# Autodesk Inventor assembly: Corpo2-3
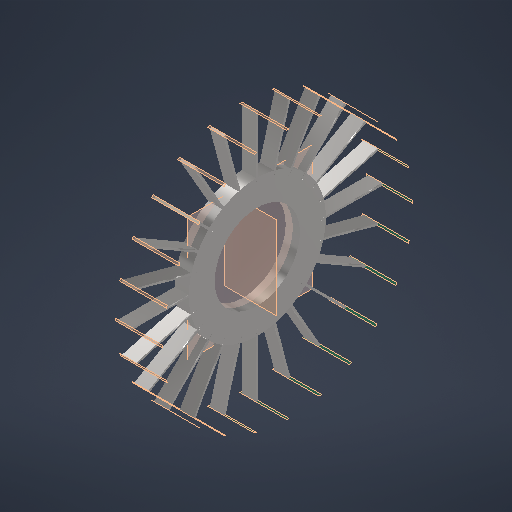
[picture p0: Inventor's stored thumbnail of the model, 512x512]
Saved by Autodesk Inventor 2026.2 (Build 302298010, 298A)
## iProperties
Created: 2026-05-01
Part Number: Corpo2-3
Document SubType Name: Assembly
Designer: Yan
Author: Yan
## Documents named in this file (3)
- C:\Users\Yan\Desktop\Turbina\Corpo2-3.iam
- C:\Users\Yan\Desktop\Turbina\CorpoDiscoPaleSatdio2-3-DimensioniAprossimate.ipt
- C:\Users\Yan\Desktop\Turbina\PalaCorpoStadio2-3.ipt
## Components (25 placed, 2 different names)
1. CorpoDiscoPaleSatdio2-3-DimensioniAprossimate:1 — Mate:1, Mate:2, Mate:3, Mate:4, Mate:5, Mate:6, Mate:7, Mate:8, Mate:9, Mate:10, Mate:11, Mate:12, Mate:13, Mate:14, Mate:15, Mate:16, Mate:17, Mate:18, Mate:19, Mate:20, Mate:21, Mate:22, Mate:23, Mate:24, Mate:25, Mate:26, Mate:27, Mate:28, Mate:29, Mate:30, Mate:31, Mate:32, Mate:33, Mate:34, Mate:35, Mate:36, Mate:37, Mate:38, Mate:39, Mate:40, Mate:41, Mate:42, Mate:43, Mate:44, Mate:45, Mate:46, Mate:47, Mate:48, Mate:49, Mate:50, Mate:51, Flush:1, Flush:2, Flush:3, Flush:4, Flush:5, Flush:6, Flush:7, Flush:8, Flush:9, Flush:10, Flush:11, Flush:12, Flush:13, Flush:14, Flush:15, Flush:16, Flush:17, Flush:18, Flush:19, Flush:20, Flush:21, Flush:22, Flush:23, Flush:24, Flush:25
2. PalaCorpoStadio2-3:1 — Mate:13, Mate:48, Flush:21
3. PalaCorpoStadio2-3:2 — Mate:14, Mate:47, Flush:22
4. PalaCorpoStadio2-3:3 — Mate:15, Mate:46, Flush:23
5. PalaCorpoStadio2-3:4 — Mate:16, Mate:45, Flush:24
6. PalaCorpoStadio2-3:5 — Mate:17, Mate:44, Flush:17
7. PalaCorpoStadio2-3:6 — Mate:18, Mate:43, Flush:16
8. PalaCorpoStadio2-3:7 — Mate:19, Mate:39, Flush:14
9. PalaCorpoStadio2-3:8 — Mate:20, Mate:40, Flush:15
10. PalaCorpoStadio2-3:9 — Mate:21, Mate:38, Flush:12
11. PalaCorpoStadio2-3:10 — Mate:22, Mate:37, Flush:11
12. PalaCorpoStadio2-3:11 — Mate:41, Mate:42, Flush:13
13. PalaCorpoStadio2-3:12 — Mate:23, Mate:36, Flush:10
14. PalaCorpoStadio2-3:13 — Mate:1, Mate:34, Flush:8
15. PalaCorpoStadio2-3:14 — Mate:2, Mate:32, Flush:6
16. PalaCorpoStadio2-3:15 — Mate:3, Mate:33, Flush:7
17. PalaCorpoStadio2-3:16 — Mate:4, Mate:35, Flush:9
18. PalaCorpoStadio2-3:17 — Mate:5, Mate:31, Flush:5
19. PalaCorpoStadio2-3:18 — Mate:6, Mate:30, Flush:4
20. PalaCorpoStadio2-3:19 — Mate:7, Mate:29, Flush:3
21. PalaCorpoStadio2-3:20 — Mate:8, Mate:24, Flush:2
22. PalaCorpoStadio2-3:21 — Mate:9, Mate:25, Flush:1, Flush:25
23. PalaCorpoStadio2-3:22 — Mate:10, Mate:26, Mate:51, Flush:18
24. PalaCorpoStadio2-3:23 — Mate:11, Mate:27, Mate:50, Flush:19
25. PalaCorpoStadio2-3:24 — Mate:12, Mate:28, Mate:49, Flush:20
## Relationships (76: Mate 51, Flush 25)
- Mate:1: CorpoDiscoPaleSatdio2-3-DimensioniAprossimate:1 ↔ PalaCorpoStadio2-3:13
- Mate:2: CorpoDiscoPaleSatdio2-3-DimensioniAprossimate:1 ↔ PalaCorpoStadio2-3:14
- Mate:3: CorpoDiscoPaleSatdio2-3-DimensioniAprossimate:1 ↔ PalaCorpoStadio2-3:15
- Mate:4: CorpoDiscoPaleSatdio2-3-DimensioniAprossimate:1 ↔ PalaCorpoStadio2-3:16
- Mate:5: CorpoDiscoPaleSatdio2-3-DimensioniAprossimate:1 ↔ PalaCorpoStadio2-3:17
- Mate:6: CorpoDiscoPaleSatdio2-3-DimensioniAprossimate:1 ↔ PalaCorpoStadio2-3:18
- Mate:7: CorpoDiscoPaleSatdio2-3-DimensioniAprossimate:1 ↔ PalaCorpoStadio2-3:19
- Mate:8: CorpoDiscoPaleSatdio2-3-DimensioniAprossimate:1 ↔ PalaCorpoStadio2-3:20
- Mate:9: CorpoDiscoPaleSatdio2-3-DimensioniAprossimate:1 ↔ PalaCorpoStadio2-3:21
- Mate:10: CorpoDiscoPaleSatdio2-3-DimensioniAprossimate:1 ↔ PalaCorpoStadio2-3:22
- Mate:11: CorpoDiscoPaleSatdio2-3-DimensioniAprossimate:1 ↔ PalaCorpoStadio2-3:23
- Mate:12: CorpoDiscoPaleSatdio2-3-DimensioniAprossimate:1 ↔ PalaCorpoStadio2-3:24
- Mate:13: CorpoDiscoPaleSatdio2-3-DimensioniAprossimate:1 ↔ PalaCorpoStadio2-3:1
- Mate:14: CorpoDiscoPaleSatdio2-3-DimensioniAprossimate:1 ↔ PalaCorpoStadio2-3:2
- Mate:15: CorpoDiscoPaleSatdio2-3-DimensioniAprossimate:1 ↔ PalaCorpoStadio2-3:3
- Mate:16: CorpoDiscoPaleSatdio2-3-DimensioniAprossimate:1 ↔ PalaCorpoStadio2-3:4
- Mate:17: CorpoDiscoPaleSatdio2-3-DimensioniAprossimate:1 ↔ PalaCorpoStadio2-3:5
- Mate:18: CorpoDiscoPaleSatdio2-3-DimensioniAprossimate:1 ↔ PalaCorpoStadio2-3:6
- Mate:19: CorpoDiscoPaleSatdio2-3-DimensioniAprossimate:1 ↔ PalaCorpoStadio2-3:7
- Mate:20: CorpoDiscoPaleSatdio2-3-DimensioniAprossimate:1 ↔ PalaCorpoStadio2-3:8
- Mate:21: CorpoDiscoPaleSatdio2-3-DimensioniAprossimate:1 ↔ PalaCorpoStadio2-3:9
- Mate:22: CorpoDiscoPaleSatdio2-3-DimensioniAprossimate:1 ↔ PalaCorpoStadio2-3:10
- Mate:23: CorpoDiscoPaleSatdio2-3-DimensioniAprossimate:1 ↔ PalaCorpoStadio2-3:12
- Mate:24: CorpoDiscoPaleSatdio2-3-DimensioniAprossimate:1 ↔ PalaCorpoStadio2-3:20
- Mate:25: CorpoDiscoPaleSatdio2-3-DimensioniAprossimate:1 ↔ PalaCorpoStadio2-3:21
- Mate:26: CorpoDiscoPaleSatdio2-3-DimensioniAprossimate:1 ↔ PalaCorpoStadio2-3:22
- Mate:27: CorpoDiscoPaleSatdio2-3-DimensioniAprossimate:1 ↔ PalaCorpoStadio2-3:23
- Mate:28: CorpoDiscoPaleSatdio2-3-DimensioniAprossimate:1 ↔ PalaCorpoStadio2-3:24
- Mate:29: CorpoDiscoPaleSatdio2-3-DimensioniAprossimate:1 ↔ PalaCorpoStadio2-3:19
- Mate:30: CorpoDiscoPaleSatdio2-3-DimensioniAprossimate:1 ↔ PalaCorpoStadio2-3:18
- Mate:31: CorpoDiscoPaleSatdio2-3-DimensioniAprossimate:1 ↔ PalaCorpoStadio2-3:17
- Mate:32: CorpoDiscoPaleSatdio2-3-DimensioniAprossimate:1 ↔ PalaCorpoStadio2-3:14
- Mate:33: CorpoDiscoPaleSatdio2-3-DimensioniAprossimate:1 ↔ PalaCorpoStadio2-3:15
- Mate:34: CorpoDiscoPaleSatdio2-3-DimensioniAprossimate:1 ↔ PalaCorpoStadio2-3:13
- Mate:35: CorpoDiscoPaleSatdio2-3-DimensioniAprossimate:1 ↔ PalaCorpoStadio2-3:16
- Mate:36: CorpoDiscoPaleSatdio2-3-DimensioniAprossimate:1 ↔ PalaCorpoStadio2-3:12
- Mate:37: CorpoDiscoPaleSatdio2-3-DimensioniAprossimate:1 ↔ PalaCorpoStadio2-3:10
- Mate:38: CorpoDiscoPaleSatdio2-3-DimensioniAprossimate:1 ↔ PalaCorpoStadio2-3:9
- Mate:39: CorpoDiscoPaleSatdio2-3-DimensioniAprossimate:1 ↔ PalaCorpoStadio2-3:7
- Mate:40: CorpoDiscoPaleSatdio2-3-DimensioniAprossimate:1 ↔ PalaCorpoStadio2-3:8
- Mate:41: CorpoDiscoPaleSatdio2-3-DimensioniAprossimate:1 ↔ PalaCorpoStadio2-3:11
- Mate:42: CorpoDiscoPaleSatdio2-3-DimensioniAprossimate:1 ↔ PalaCorpoStadio2-3:11
- Mate:43: CorpoDiscoPaleSatdio2-3-DimensioniAprossimate:1 ↔ PalaCorpoStadio2-3:6
- Mate:44: CorpoDiscoPaleSatdio2-3-DimensioniAprossimate:1 ↔ PalaCorpoStadio2-3:5
- Mate:45: CorpoDiscoPaleSatdio2-3-DimensioniAprossimate:1 ↔ PalaCorpoStadio2-3:4
- Mate:46: CorpoDiscoPaleSatdio2-3-DimensioniAprossimate:1 ↔ PalaCorpoStadio2-3:3
- Mate:47: CorpoDiscoPaleSatdio2-3-DimensioniAprossimate:1 ↔ PalaCorpoStadio2-3:2
- Mate:48: CorpoDiscoPaleSatdio2-3-DimensioniAprossimate:1 ↔ PalaCorpoStadio2-3:1
- Mate:49: CorpoDiscoPaleSatdio2-3-DimensioniAprossimate:1 ↔ PalaCorpoStadio2-3:24
- Mate:50: CorpoDiscoPaleSatdio2-3-DimensioniAprossimate:1 ↔ PalaCorpoStadio2-3:23
- Mate:51: CorpoDiscoPaleSatdio2-3-DimensioniAprossimate:1 ↔ PalaCorpoStadio2-3:22
- Flush:1: CorpoDiscoPaleSatdio2-3-DimensioniAprossimate:1 ↔ PalaCorpoStadio2-3:21
- Flush:2: CorpoDiscoPaleSatdio2-3-DimensioniAprossimate:1 ↔ PalaCorpoStadio2-3:20
- Flush:3: CorpoDiscoPaleSatdio2-3-DimensioniAprossimate:1 ↔ PalaCorpoStadio2-3:19
- Flush:4: CorpoDiscoPaleSatdio2-3-DimensioniAprossimate:1 ↔ PalaCorpoStadio2-3:18
- Flush:5: CorpoDiscoPaleSatdio2-3-DimensioniAprossimate:1 ↔ PalaCorpoStadio2-3:17
- Flush:6: CorpoDiscoPaleSatdio2-3-DimensioniAprossimate:1 ↔ PalaCorpoStadio2-3:14
- Flush:7: CorpoDiscoPaleSatdio2-3-DimensioniAprossimate:1 ↔ PalaCorpoStadio2-3:15
- Flush:8: CorpoDiscoPaleSatdio2-3-DimensioniAprossimate:1 ↔ PalaCorpoStadio2-3:13
- Flush:9: CorpoDiscoPaleSatdio2-3-DimensioniAprossimate:1 ↔ PalaCorpoStadio2-3:16
- Flush:10: CorpoDiscoPaleSatdio2-3-DimensioniAprossimate:1 ↔ PalaCorpoStadio2-3:12
- Flush:11: CorpoDiscoPaleSatdio2-3-DimensioniAprossimate:1 ↔ PalaCorpoStadio2-3:10
- Flush:12: CorpoDiscoPaleSatdio2-3-DimensioniAprossimate:1 ↔ PalaCorpoStadio2-3:9
- Flush:13: CorpoDiscoPaleSatdio2-3-DimensioniAprossimate:1 ↔ PalaCorpoStadio2-3:11
- Flush:14: CorpoDiscoPaleSatdio2-3-DimensioniAprossimate:1 ↔ PalaCorpoStadio2-3:7
- Flush:15: CorpoDiscoPaleSatdio2-3-DimensioniAprossimate:1 ↔ PalaCorpoStadio2-3:8
- Flush:16: CorpoDiscoPaleSatdio2-3-DimensioniAprossimate:1 ↔ PalaCorpoStadio2-3:6
- Flush:17: CorpoDiscoPaleSatdio2-3-DimensioniAprossimate:1 ↔ PalaCorpoStadio2-3:5
- Flush:18: CorpoDiscoPaleSatdio2-3-DimensioniAprossimate:1 ↔ PalaCorpoStadio2-3:22
- Flush:19: CorpoDiscoPaleSatdio2-3-DimensioniAprossimate:1 ↔ PalaCorpoStadio2-3:23
- Flush:20: CorpoDiscoPaleSatdio2-3-DimensioniAprossimate:1 ↔ PalaCorpoStadio2-3:24
- Flush:21: CorpoDiscoPaleSatdio2-3-DimensioniAprossimate:1 ↔ PalaCorpoStadio2-3:1
- Flush:22: CorpoDiscoPaleSatdio2-3-DimensioniAprossimate:1 ↔ PalaCorpoStadio2-3:2
- Flush:23: CorpoDiscoPaleSatdio2-3-DimensioniAprossimate:1 ↔ PalaCorpoStadio2-3:3
- Flush:24: CorpoDiscoPaleSatdio2-3-DimensioniAprossimate:1 ↔ PalaCorpoStadio2-3:4
- Flush:25: CorpoDiscoPaleSatdio2-3-DimensioniAprossimate:1 ↔ PalaCorpoStadio2-3:21
